# Autodesk Inventor assembly: RSX Assembly
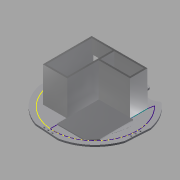
[picture p0: Inventor's stored thumbnail of the model, 180x180]
Saved by Autodesk Inventor 2017 (Build 210142000, 142)
## iProperties
Created: 2016-10-28
Part Number: RSX Assembly
Document SubType Name: Assembly
Designer: eschr_000
Author: eschr_000
## Documents named in this file (11)
- C:\Users\qupec\Desktop\UMD Near Space\STAR\CAD\Mechanical\CapTech\RSX Assembly.iam
- C:\Users\qupec\Desktop\UMD Near Space\STAR\CAD\Mechanical\CapTech\RSX Structure.ipt
- C:\Users\qupec\Desktop\UMD Near Space\STAR\CAD\Mechanical\CapTech\VR Camera.ipt
- C:\Users\qupec\Desktop\UMD Near Space\STAR\CAD\Mechanical\CapTech\Antenna.ipt
- C:\Users\qupec\Desktop\UMD Near Space\STAR\CAD\Mechanical\CapTech\Pi Zero.iam
- C:\Users\qupec\Desktop\UMD Near Space\STAR\CAD\Mechanical\CapTech\Hermes Cube.ipt
- C:\Users\qupec\Desktop\UMD Near Space\STAR\CAD\Mechanical\CapTech\VR Camera Dome.ipt
- C:\Users\qupec\Desktop\UMD Near Space\STAR\CAD\Mechanical\CapTech\Keep Out RSX Deck.ipt
- C:\Users\qupec\Desktop\UMD Near Space\STAR\CAD\Mechanical\CapTech\RSX Deck.ipt
- C:\Users\qupec\Desktop\UMD Near Space\STAR\CAD\Mechanical\CapTech\RSX Top.ipt
- C:\Users\qupec\Desktop\UMD Near Space\STAR\CAD\Mechanical\Base Plate Mk 2.ipt
## Components (10 placed, 10 different names)
1. RSX Structure:1 — Mate:5, Mate:6, Mate:7, Mate:8, Mate:10, Flush:1, Mate:13, Mate:16, Symmetry:1, Mate:22, Mate:23, Mate:25, Mate:26, Mate:29, Mate:30, Mate:31, Mate:32, Mate:33, Mate:36, Mate:37, Mate:38
2. VR Camera:1 — Flush:1, Mate:13, Mate:14, Mate:15, Mate:25
3. Antenna:1 — Mate:6
4. Pi Zero:1 [sub-assembly] — Mate:5, Mate:7, Mate:8, Mate:32
5. Hermes Cube:1 — Mate:10, Symmetry:1, Mate:22, Mate:23
6. VR Camera Dome:1 — Mate:14, Mate:15
7. Keep Out RSX Deck:1 — Mate:16
8. RSX Top:1 — Mate:29, Mate:30, Mate:31
9. RSX Deck:1 — Mate:26, Mate:33, Mate:35, Mate:38
10. Base Plate Mk 2:1 — Mate:35, Mate:36, Mate:37
## Relationships (24: Mate 22, Flush 1, Symmetry 1)
- Mate:5: RSX Structure:1 ↔ Pi Zero:1
- Mate:6: RSX Structure:1 ↔ Antenna:1
- Mate:7: RSX Structure:1 ↔ Pi Zero:1
- Mate:8: RSX Structure:1 ↔ Pi Zero:1
- Mate:10: RSX Structure:1 ↔ Hermes Cube:1
- Flush:1: RSX Structure:1 ↔ VR Camera:1
- Mate:13 (28 mm): RSX Structure:1 ↔ VR Camera:1
- Mate:14: VR Camera:1 ↔ VR Camera Dome:1
- Mate:15: VR Camera:1 ↔ VR Camera Dome:1
- Mate:16: RSX Structure:1 ↔ Keep Out RSX Deck:1
- Symmetry:1: RSX Structure:1 ↔ Hermes Cube:1
- Mate:22: RSX Structure:1 ↔ Hermes Cube:1
- Mate:23: RSX Structure:1 ↔ Hermes Cube:1
- Mate:25 (38.1 mm): RSX Structure:1 ↔ VR Camera:1
- Mate:26: RSX Structure:1 ↔ RSX Deck:1
- Mate:29: RSX Structure:1 ↔ RSX Top:1
- Mate:30: RSX Structure:1 ↔ RSX Top:1
- Mate:31: RSX Structure:1 ↔ RSX Top:1
- Mate:32: RSX Structure:1 ↔ Pi Zero:1
- Mate:33: RSX Structure:1 ↔ RSX Deck:1
- Mate:35: RSX Deck:1 ↔ Base Plate Mk 2:1
- Mate:36: RSX Structure:1 ↔ Base Plate Mk 2:1
- Mate:37: RSX Structure:1 ↔ Base Plate Mk 2:1
- Mate:38: RSX Structure:1 ↔ RSX Deck:1
